# Autodesk Inventor assembly: Dribbler-3-gears
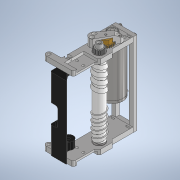
[picture p0: Inventor's stored thumbnail of the model, 180x180]
Saved by Autodesk Inventor 2020.2 (Build 242310000, 310)
## iProperties
Created: 2021-02-21
Part Number: Dribbler-3-gears
Document SubType Name: Assembly
Designer: Acer
Author: Acer
## Documents named in this file (16)
- G:\Meu Drive\RobôCIn\Mecânica\SSL\2021\vRoboCup2021\dribbler-3-gears\Dribbler-3-gears.iam
- G:\Meu Drive\RobôCIn\Mecânica\SSL\2021\vRoboCup2021\dribbler-3-gears\PartA_3D.ipt
- G:\Meu Drive\RobôCIn\Mecânica\SSL\2021\vRoboCup2021\dribbler-3-gears\Kugellager 685-ZZ-C3.ipt
- G:\Meu Drive\RobôCIn\Mecânica\SSL\2021\vRoboCup2021\dribbler-3-gears\Eixo.ipt
- G:\Meu Drive\RobôCIn\Mecânica\SSL\2021\vRoboCup2021\dribbler-3-gears\MaxonECmax22-25W.ipt
- G:\Meu Drive\RobôCIn\Mecânica\SSL\2021\vRoboCup2021\dribbler-3-gears\gear_z18_21101800(modified).ipt
- G:\Meu Drive\RobôCIn\Mecânica\SSL\2021\vRoboCup2021\dribbler-3-gears\gear_z18_21101800_di3.ipt
- G:\Meu Drive\RobôCIn\Mecânica\SSL\2021\vRoboCup2021\dribbler-3-gears\PartD_3D.ipt
- G:\Meu Drive\RobôCIn\Mecânica\SSL\2021\vRoboCup2021\dribbler-3-gears\Dribblerschnecke.ipt
- G:\Meu Drive\RobôCIn\Mecânica\SSL\2021\vRoboCup2021\dribbler-3-gears\PartC_3D.ipt
- G:\Meu Drive\RobôCIn\Mecânica\SSL\2021\vRoboCup2021\dribbler-3-gears\PartB_3D.ipt
- G:\Meu Drive\RobôCIn\Mecânica\SSL\2021\vRoboCup2021\dribbler-3-gears\ChipKicker_v2020_3D.ipt
- G:\Meu Drive\RobôCIn\Mecânica\SSL\2021\vRoboCup2021\dribbler-3-gears\Middle_Gear.iam
- C:\Users\Acer\Documents\Inventor\Content Center Files\R2020\en-US\DIN EN ISO 4032\DIN EN ISO 4032 - M2.ipt
- C:\Users\Acer\Documents\Inventor\Content Center Files\R2020\en-US\DIN 84\DIN 84 - M2 x 8.ipt
- C:\Users\Acer\Documents\Inventor\Content Center Files\R2020\en-US\DIN 84\DIN 84 - M2 x 6.ipt
## Components (22 placed, 14 different names)
1. PartA_3D:1 — Mate:1, Flush:1, Mate:4, Mate:5, Mate:7, Mate:11, Mate:12, Mate:13, Mate:15, Mate:16, Mate:17, Mate:18, Mate:27, Flush:4, Angle:1, Mate:28, Flush:5, Angle:2, Mate:29, Flush:6, Angle:3
2. Kugellager 685-ZZ-C3:1 — Mate:1, Flush:1, Mate:2, Mate:3
3. Eixo:1 — Mate:2, Mate:3, Mate:6, Mate:14, Rotation:3, Rotation:4, Mate:22
4. MaxonECmax22-25W:1 — Mate:4, Mate:5, Mate:8, Flush:2
5. Ritzel z=18:1 — Mate:6, Mate:7, Rotation:4, Rotation:6
6. Ritzel z=18:2 — Mate:8, Flush:2, Rotation:5
7. PartD_3D:1 — Mate:11, Mate:12, Mate:13, Mate:25, Mate:30, Mate:31, Mate:32, Mate:39
8. Dribblerschnecke:1 — Mate:14, Mate:15, Rotation:3
9. PartC_3D:1 — Mate:16, Mate:17, Mate:18, Mate:19, Mate:20, Mate:21, Mate:33, Mate:34, Mate:35, Mate:36, Mate:37, Mate:38
10. PartB_3D:1 — Mate:19, Mate:20, Mate:21, Flush:3, Mate:23, Mate:24
11. Kugellager 685-ZZ-C3:2 — Mate:22, Flush:3
12. ChipKicker_v2020_3D:1 — Mate:23, Mate:24
13. Middle_Gear:1 [sub-assembly] — Mate:25, Rotation:5, Rotation:6, Mate:39
14. DIN EN ISO 4032 M2:1 — Mate:29, Flush:6, Angle:3, Flush:9
15. DIN EN ISO 4032 M2:2 — Mate:28, Flush:5, Angle:2, Flush:8
16. DIN EN ISO 4032 M2:3 — Mate:27, Flush:4, Angle:1, Flush:7
17. DIN 84 - replaced by DIN EN ISO 1207 M2 x 8:1 — Mate:30, Flush:7
18. DIN 84 - replaced by DIN EN ISO 1207 M2 x 8:2 — Mate:31, Flush:8
19. DIN 84 - replaced by DIN EN ISO 1207 M2 x 8:3 — Mate:32, Flush:9
20. DIN 84 - replaced by DIN EN ISO 1207 M2 x 6:1 — Mate:33, Mate:34
21. DIN 84 - replaced by DIN EN ISO 1207 M2 x 6:2 — Mate:35, Mate:36
22. DIN 84 - replaced by DIN EN ISO 1207 M2 x 8:4 — Mate:37, Mate:38
## Relationships (52: Mate 36, Flush 9, RelateRotation 4, Angle 3)
- Mate:1: PartA_3D:1 ↔ Kugellager 685-ZZ-C3:1
- Flush:1: PartA_3D:1 ↔ Kugellager 685-ZZ-C3:1
- Mate:2: Kugellager 685-ZZ-C3:1 ↔ Eixo:1
- Mate:3: Kugellager 685-ZZ-C3:1 ↔ Eixo:1
- Mate:4: PartA_3D:1 ↔ MaxonECmax22-25W:1
- Mate:5: PartA_3D:1 ↔ MaxonECmax22-25W:1
- Mate:6: Eixo:1 ↔ Ritzel z=18:1
- Mate:7: PartA_3D:1 ↔ Ritzel z=18:1
- Mate:8: MaxonECmax22-25W:1 ↔ Ritzel z=18:2
- Flush:2 (1 mm): MaxonECmax22-25W:1 ↔ Ritzel z=18:2
- Mate:11: PartA_3D:1 ↔ PartD_3D:1
- Mate:12: PartA_3D:1 ↔ PartD_3D:1
- Mate:13: PartA_3D:1 ↔ PartD_3D:1
- Mate:14: Eixo:1 ↔ Dribblerschnecke:1
- Mate:15 (2 mm): PartA_3D:1 ↔ Dribblerschnecke:1
- Rotation:3 [RelateRotation] (1 ul): Eixo:1 ↔ Dribblerschnecke:1
- Rotation:4 [RelateRotation] (1.25 ul): Eixo:1 ↔ Ritzel z=18:1
- Mate:16: PartA_3D:1 ↔ PartC_3D:1
- Mate:17: PartA_3D:1 ↔ PartC_3D:1
- Mate:18: PartA_3D:1 ↔ PartC_3D:1
- Mate:19: PartC_3D:1 ↔ PartB_3D:1
- Mate:20: PartC_3D:1 ↔ PartB_3D:1
- Mate:21: PartC_3D:1 ↔ PartB_3D:1
- Mate:22: Eixo:1 ↔ Kugellager 685-ZZ-C3:2
- Flush:3: PartB_3D:1 ↔ Kugellager 685-ZZ-C3:2
- Mate:23: PartB_3D:1 ↔ ChipKicker_v2020_3D:1
- Mate:24 (0.5 mm): PartB_3D:1 ↔ ChipKicker_v2020_3D:1
- Mate:25: PartD_3D:1 ↔ Middle_Gear:1
- Rotation:5 [RelateRotation] (0.6923 ul): Ritzel z=18:2 ↔ Middle_Gear:1
- Rotation:6 [RelateRotation] (1.444 ul): Ritzel z=18:1 ↔ Middle_Gear:1
- Mate:27: PartA_3D:1 ↔ DIN EN ISO 4032 M2:3
- Flush:4: PartA_3D:1 ↔ DIN EN ISO 4032 M2:3
- Angle:1 (0 deg): PartA_3D:1 ↔ DIN EN ISO 4032 M2:3
- Mate:28: PartA_3D:1 ↔ DIN EN ISO 4032 M2:2
- Flush:5: PartA_3D:1 ↔ DIN EN ISO 4032 M2:2
- Angle:2 (0 deg): PartA_3D:1 ↔ DIN EN ISO 4032 M2:2
- Mate:29: PartA_3D:1 ↔ DIN EN ISO 4032 M2:1
- Flush:6: PartA_3D:1 ↔ DIN EN ISO 4032 M2:1
- Angle:3 (0 deg): PartA_3D:1 ↔ DIN EN ISO 4032 M2:1
- Mate:30: PartD_3D:1 ↔ DIN 84 - replaced by DIN EN ISO 1207 M2 x 8:1
- Mate:31: PartD_3D:1 ↔ DIN 84 - replaced by DIN EN ISO 1207 M2 x 8:2
- Mate:32: PartD_3D:1 ↔ DIN 84 - replaced by DIN EN ISO 1207 M2 x 8:3
- Flush:7 (0.2 mm): DIN EN ISO 4032 M2:3 ↔ DIN 84 - replaced by DIN EN ISO 1207 M2 x 8:1
- Flush:8 (0.2 mm): DIN EN ISO 4032 M2:2 ↔ DIN 84 - replaced by DIN EN ISO 1207 M2 x 8:2
- Flush:9 (0.2 mm): DIN EN ISO 4032 M2:1 ↔ DIN 84 - replaced by DIN EN ISO 1207 M2 x 8:3
- Mate:33: PartC_3D:1 ↔ DIN 84 - replaced by DIN EN ISO 1207 M2 x 6:1
- Mate:34: PartC_3D:1 ↔ DIN 84 - replaced by DIN EN ISO 1207 M2 x 6:1
- Mate:35: PartC_3D:1 ↔ DIN 84 - replaced by DIN EN ISO 1207 M2 x 6:2
- Mate:36: PartC_3D:1 ↔ DIN 84 - replaced by DIN EN ISO 1207 M2 x 6:2
- Mate:37: PartC_3D:1 ↔ DIN 84 - replaced by DIN EN ISO 1207 M2 x 8:4
- Mate:38 (1.2 mm): PartC_3D:1 ↔ DIN 84 - replaced by DIN EN ISO 1207 M2 x 8:4
- Mate:39 (0.075 mm): PartD_3D:1 ↔ Middle_Gear:1
